# Autodesk Inventor assembly: Сборка1
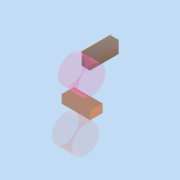
[picture p0: Inventor's stored thumbnail of the model, 180x180]
Saved by Autodesk Inventor 2019 (Build 230136000, 136)
## iProperties
Created: 2021-02-11
Part Number: Сборка1
Material: Типовые
Document SubType Name: Assembly
Designer: Kurbatova
Author: Kurbatova
## Documents named in this file (3)
- C:\Users\Kurbatova\source\LW2020\lw_2021\LW_SAPR\Сборки\Сборка1.iam
- C:\Users\Kurbatova\source\LW2020\lw_2021\LW_SAPR\Детали\Деталь2.ipt
- C:\Users\Kurbatova\source\LW2020\lw_2021\LW_SAPR\Детали\Деталь1.ipt
## Components (4 placed, 2 different names)
1. Деталь1:1
2. Деталь2:2 — Касательность:1
3. Деталь1:2 — Касательность:1
4. Деталь2:3
## Relationships (1: Tangent 1)
- Касательность:1 [Tangent]: Деталь2:2 ↔ Деталь1:2
